# Autodesk Inventor assembly: Shoulder
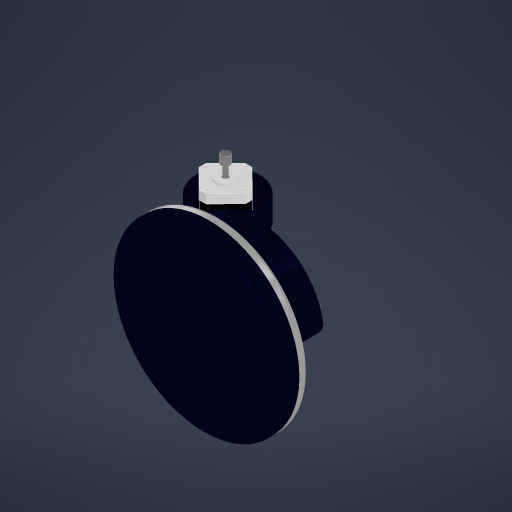
[picture p0: Inventor's stored thumbnail of the model, 512x512]
Saved by Autodesk Inventor 2023 (Build 270158000, 158)
## iProperties
Created: 2023-04-07
Part Number: Shoulder
Document SubType Name: Assembly
Designer: vatdu
Author: vatdu
## Documents named in this file (5)
- C:\Users\vatdu\Desktop\CRYSTAL MARK II\Shoulder\Shoulder.iam
- C:\Users\vatdu\Desktop\CRYSTAL MARK II\Shoulder\Rotating Plate.ipt
- C:\Users\vatdu\Desktop\CRYSTAL MARK II\Components\Stepper Motor.ipt
- C:\Users\vatdu\Desktop\CRYSTAL MARK II\Shoulder\Motor Cover.ipt
- C:\Users\vatdu\Desktop\CRYSTAL MARK II\Shoulder\Arm Extention.ipt
## Components (5 placed, 4 different names)
1. Rotating Plate:1 — Rotational:1
2. Stepper Motor:1 — Rotational:2
3. Motor Cover:1 — Rotational:1
4. Arm Extention:1 — Rotational:2, Rigid:1
5. Stepper Motor:2 — Rigid:1
## Relationships (3: RevoluteJoint 2, WeldJoint 1)
- Rotational:1 [RevoluteJoint]: Rotating Plate:1 ↔ Motor Cover:1
- Rotational:2 [RevoluteJoint]: Stepper Motor:1 ↔ Arm Extention:1
- Rigid:1 [WeldJoint]: Arm Extention:1 ↔ Stepper Motor:2
